# Autodesk Inventor assembly: FirstAssembly
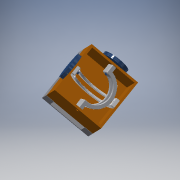
[picture p0: Inventor's stored thumbnail of the model, 180x180]
Saved by Autodesk Inventor 2017 (Build 210142000, 142)
## iProperties
Created: 2017-02-25
Part Number: FirstAssembly
Document SubType Name: Assembly
Designer: aribu
Author: aribu
## Documents named in this file (7)
- C:\Users\aribu\Dropbox\Kettering\CE-490 CE Capstone\GitHub\Hardware\Inventor Files\V2\FirstAssembly.iam
- C:\Users\aribu\Dropbox\Kettering\CE-490 CE Capstone\GitHub\Hardware\Inventor Files\V2\BottomCircleArm.ipt
- C:\Users\aribu\Dropbox\Kettering\CE-490 CE Capstone\GitHub\Hardware\Inventor Files\V2\Box.ipt
- C:\Users\aribu\Dropbox\Kettering\CE-490 CE Capstone\GitHub\Hardware\Inventor Files\V2\FalseFloor.ipt
- C:\Users\aribu\Dropbox\Kettering\CE-490 CE Capstone\GitHub\Hardware\Inventor Files\V2\TopCircleArm.ipt
- C:\Users\aribu\Dropbox\Kettering\CE-490 CE Capstone\GitHub\Hardware\Inventor Files\V2\PulleyAdapter.ipt
- C:\Users\aribu\Dropbox\Kettering\CE-490 CE Capstone\GitHub\Hardware\Inventor Files\V2\PulleyAdapterLong.ipt
## Components (6 placed, 6 different names)
1. BottomCircleArm:1 — Rotational:2, Mate:2, Mate:3
2. Box:1 — Mate:1, Flush:1, Flush:2, Rotational:1, Rotational:2, Mate:4, Mate:7
3. FalseFloor:1 — Mate:1, Flush:1, Flush:2
4. TopCircleArm:1 — Rotational:1, Mate:5, Mate:6
5. PulleyAdapter:2 — Mate:2, Mate:3, Mate:4
6. PulleyAdapterLong:1 — Mate:5, Mate:6, Mate:7
## Relationships (11: Mate 7, Flush 2, RevoluteJoint 2)
- Mate:1: Box:1 ↔ FalseFloor:1
- Flush:1: Box:1 ↔ FalseFloor:1
- Flush:2: Box:1 ↔ FalseFloor:1
- Rotational:1 [RevoluteJoint]: Box:1 ↔ TopCircleArm:1
- Rotational:2 [RevoluteJoint]: BottomCircleArm:1 ↔ Box:1
- Mate:2: BottomCircleArm:1 ↔ PulleyAdapter:2
- Mate:3: BottomCircleArm:1 ↔ PulleyAdapter:2
- Mate:4 (0.2 mm): Box:1 ↔ PulleyAdapter:2
- Mate:5: TopCircleArm:1 ↔ PulleyAdapterLong:1
- Mate:6: TopCircleArm:1 ↔ PulleyAdapterLong:1
- Mate:7 (0.2 mm): Box:1 ↔ PulleyAdapterLong:1
